# Autodesk Inventor assembly: Assembly1
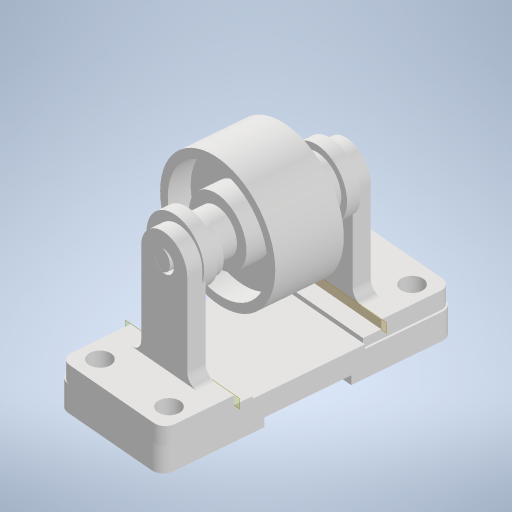
[picture p0: Inventor's stored thumbnail of the model, 512x512]
Saved by Autodesk Inventor 2024 (Build 280153000, 153)
## iProperties
Created: 2024-06-04
Part Number: Assembly1
Document SubType Name: Assembly
Designer: Ricsi
Author: Ricsi
## Documents named in this file (6)
- D:\Dokumentumok\VTS\Gépelemek 1\sddfdsfsdf\Assembly1.iam
- D:\Dokumentumok\VTS\Gépelemek 1\sddfdsfsdf\burc.ipt
- D:\Dokumentumok\VTS\Gépelemek 1\sddfdsfsdf\kasnak.ipt
- D:\Dokumentumok\VTS\Gépelemek 1\sddfdsfsdf\mi.ipt
- D:\Dokumentumok\VTS\Gépelemek 1\sddfdsfsdf\ttab.ipt
- D:\Dokumentumok\VTS\Gépelemek 1\sddfdsfsdf\yatak.ipt
## Components (7 placed, 5 different names)
1. kasnak:1 — Mate:3, Insert:6
2. mi:1 — Insert:5, Mate:3, Mate:4
3. ttab:1 — Mate:1, Insert:1, Insert:2, Mate:2, Insert:3, Insert:4
4. yatak:1 — Mate:1, Insert:1, Insert:2, Insert:5
5. yatak:2 — Mate:2, Insert:3, Insert:4
6. burc:1 — Mate:4
7. burc:2 — Insert:6
## Relationships (10: Insert 6, Mate 4)
- Mate:1: ttab:1 ↔ yatak:1
- Insert:1: ttab:1 ↔ yatak:1
- Insert:2: ttab:1 ↔ yatak:1
- Mate:2: ttab:1 ↔ yatak:2
- Insert:3: ttab:1 ↔ yatak:2
- Insert:4: ttab:1 ↔ yatak:2
- Insert:5: mi:1 ↔ yatak:1
- Mate:3: kasnak:1 ↔ mi:1
- Insert:6: kasnak:1 ↔ burc:2
- Mate:4: mi:1 ↔ burc:1
